# Autodesk Inventor assembly: Krasser Roboter
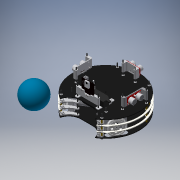
[picture p0: Inventor's stored thumbnail of the model, 180x180]
Saved by Autodesk Inventor 2018 (Build 220112000, 112)
## iProperties
Created: 2019-03-04
Part Number: Krasser Roboter
Material: Generisch
Document SubType Name: Assembly
Designer: RedBots
Mass: 1130.14 g
Surface Area: 3109.1 cm^2
Volume: 625.212 cm^3
Density: 1.80761 g/cm^3
Author: RedBots
## Documents named in this file (30)
- C:\Users\RedBots\Desktop\FinalRobot\Krasser Roboter.iam
- C:\Users\RedBots\Desktop\FinalRobot\Bodenplatine.ipt
- C:\Users\RedBots\Desktop\FinalRobot\motorhalterung 3.0.ipt
- C:\Users\RedBots\Desktop\FinalRobot\Gewindestange M3x100mm.ipt
- C:\Users\RedBots\Desktop\FinalRobot\Gewindestange M3x70mm.ipt
- C:\Users\RedBots\Desktop\FinalRobot\alu_ring_pesus.ipt
- C:\Users\RedBots\Desktop\FinalRobot\Fake Rad.ipt
- C:\Users\RedBots\Desktop\FinalRobot\Hauptplatine.ipt
- C:\Users\RedBots\Desktop\FinalRobot\Akku.ipt
- C:\Users\RedBots\Desktop\FinalRobot\Akkuhalterung.ipt
- C:\Users\RedBots\Desktop\FinalRobot\Schraube M3x8 SK.ipt
- C:\Users\RedBots\Desktop\FinalRobot\Motor\Motormaxon_PN_B7453F27107C.iam
- C:\Users\RedBots\Desktop\FinalRobot\Abstandshalter 15mm.ipt
- C:\Users\RedBots\Desktop\FinalRobot\LED 3mm.ipt
- C:\Users\RedBots\Desktop\FinalRobot\Halterung Lichtschranke rechts.ipt
- C:\Users\RedBots\Desktop\FinalRobot\Ball.ipt
- C:\Users\RedBots\Desktop\FinalRobot\Halterung Lichtschranke links.ipt
- C:\Users\RedBots\Desktop\FinalRobot\Abstandshalter 12mm.ipt
- C:\Users\RedBots\Desktop\FinalRobot\SRF08.ipt
- C:\Users\RedBots\Desktop\FinalRobot\US Halterung hinten.ipt
- C:\Users\RedBots\Desktop\FinalRobot\Pinhead 5.ipt
- C:\Users\RedBots\Desktop\FinalRobot\Schraube M3x8 LK.ipt
- C:\Users\RedBots\Desktop\FinalRobot\US Halterung rechts.ipt
- C:\Users\RedBots\Desktop\FinalRobot\US Halterung links.ipt
- C:\Users\RedBots\Desktop\FinalRobot\Pixy 2.iam
- C:\Users\RedBots\Desktop\FinalRobot\Pixy 2 Halterung.ipt
- C:\Users\RedBots\Desktop\FinalRobot\Abstandshalter US Sensor.ipt
- C:\Users\RedBots\Desktop\FinalRobot\Schraube M3x10 LK.ipt
- C:\Users\RedBots\Desktop\FinalRobot\Scheibe M3 Polyamid.ipt
- C:\Users\RedBots\Desktop\FinalRobot\Sicherungsmutter M3.ipt
## Components (131 placed, 30 different names)
1. Ball:1 — Passend:142, Passend:143
2. Abstandshalter US Sensor:1 — Passend:222, Passend:224, Passend:226
3. Abstandshalter US Sensor:2 — Passend:223, Passend:225
4. Bodenplatine:1 — Passend:16, Passend:17, Fluchtend:1, Fluchtend:2, Passend:18, Passend:19, Passend:20, Fluchtend:3, Fluchtend:4, Passend:21, Passend:22, Passend:23, Fluchtend:5, Fluchtend:6, Passend:24, Passend:25, Passend:26, Passend:27, Passend:28, Passend:29, Passend:30, Passend:31, Passend:32, Fluchtend:7, Fluchtend:8, Fluchtend:9, Fluchtend:10, Fluchtend:11, Fluchtend:12, Fluchtend:13, Fluchtend:14, Passend:100, Passend:102, Passend:105, Passend:106, Passend:143, Passend:157, Passend:158, Passend:262, Passend:263, Passend:264, Passend:265, Passend:266, Passend:267, Passend:268, Passend:269, Passend:270, Passend:271, Passend:272, Passend:273, Passend:274, Passend:275
5. Hauptplatine:1 — Passend:48, Passend:49, Passend:50, Passend:53, Passend:54, Passend:61, Passend:63, Passend:168, Passend:181, Passend:202, Passend:210, Passend:238, Passend:239, Passend:240, Passend:241, Passend:242, Passend:243, Passend:244, Passend:245, Passend:246, Passend:247, Passend:304
6. Gewindestange M3x100mm:1 — Passend:15, Passend:22, Fluchtend:6, Passend:169, Passend:233, Passend:255, Passend:284
7. Gewindestange M3x100mm:2 — Passend:14, Passend:23, Fluchtend:5, Passend:167, Passend:232, Passend:254, Passend:281
8. Gewindestange M3x100mm:8 — Passend:28, Fluchtend:8, Passend:62, Passend:128, Passend:137, Passend:140, Passend:209, Passend:250, Passend:293
9. Gewindestange M3x100mm:11 — Passend:26, Fluchtend:9, Passend:60, Passend:130, Passend:134, Passend:138, Passend:208, Passend:261, Passend:276
10. Gewindestange M3x100mm:12 — Passend:13, Passend:17, Fluchtend:2, Passend:179, Passend:235, Passend:258, Passend:292
11. Gewindestange M3x70mm:2 — Passend:12, Passend:16, Fluchtend:1, Passend:259, Passend:299
12. Gewindestange M3x100mm:14 — Passend:11, Passend:20, Fluchtend:3, Passend:203, Passend:229, Passend:251, Passend:278
13. Gewindestange M3x70mm:9 — Passend:10, Passend:19, Fluchtend:4, Passend:228, Passend:249, Passend:296
14. Gewindestange M3x70mm:1 — Passend:25, Fluchtend:10, Passend:33, Passend:36, Passend:49, Passend:86, Passend:87, Passend:112, Passend:131, Passend:135, Passend:139, Passend:234, Passend:260, Passend:298
15. Gewindestange M3x70mm:10 — Passend:29, Fluchtend:7, Passend:34, Passend:37, Passend:50, Passend:92, Passend:93, Passend:113, Passend:129, Passend:136, Passend:141, Passend:227, Passend:248, Passend:300
16. Gewindestange M3x100mm:15 — Passend:30, Fluchtend:14, Passend:94, Passend:95, Passend:114, Passend:204, Passend:230, Passend:252, Passend:280
17. Gewindestange M3x70mm:5 — Passend:32, Fluchtend:12, Passend:90, Passend:91, Passend:116, Passend:237, Passend:256, Passend:288
18. Gewindestange M3x70mm:6 — Passend:31, Fluchtend:13, Passend:96, Passend:97, Passend:117, Passend:231, Passend:253, Passend:285
19. Gewindestange M3x100mm:13 — Passend:27, Fluchtend:11, Passend:88, Passend:89, Passend:115, Passend:180, Passend:236, Passend:257, Passend:289
20. Ring unten — Passend:33, Passend:34, Passend:101, Passend:103, Passend:104, Passend:107, Passend:110, Passend:156, Passend:159
21. Ring oben — Passend:36, Passend:37, Passend:111, Passend:118, Passend:119, Passend:120, Passend:121, Passend:132, Passend:133
22. Fake Rad:1 — Tangential:2, Passend:75, Fluchtend:23
23. Fake Rad:2 — Tangential:1, Passend:70, Fluchtend:22
24. Fake Rad:3 — Passend:76, Fluchtend:24
25. Akku:1 — Passend:59, Passend:64, Fluchtend:18
26. Akkuhalterung:1 — Passend:54, Passend:62, Passend:63
27. Akkuhalterung:2 — Passend:53, Passend:59, Passend:60, Passend:61, Passend:64, Fluchtend:18
28. Motormaxon_PN_B7453F27107C:3 [sub-assembly] — Passend:68, Passend:69, Passend:70, Fluchtend:22, Passend:85
29. Motormaxon_PN_B7453F27107C:1 [sub-assembly] — Passend:71, Passend:72, Passend:75, Fluchtend:23, Passend:84
30. Motormaxon_PN_B7453F27107C:2 [sub-assembly] — Passend:73, Passend:74, Passend:76, Fluchtend:24, Passend:80, Passend:81, Passend:82, Passend:83
31. Abstandshalter 12mm:3 — Passend:86, Passend:98
32. Abstandshalter 12mm:2 — Passend:87, Passend:99
33. Abstandshalter 12mm:5 — Passend:93, Passend:109
34. Abstandshalter 12mm:6 — Passend:92, Passend:108, Passend:110
35. Abstandshalter 12mm:1 — Passend:112, Passend:122
36. Abstandshalter 12mm:4 — Passend:113, Passend:123
37. Abstandshalter 15mm:3 — Passend:97, Passend:104
38. Abstandshalter 15mm:4 — Passend:95, Passend:107, Passend:111
39. Abstandshalter 15mm:5 — Passend:96, Passend:105
40. Abstandshalter 15mm:6 — Passend:94, Passend:106
41. Abstandshalter 15mm:7 — Passend:88, Passend:101
42. Abstandshalter 15mm:8 — Passend:89, Passend:100
43. Abstandshalter 15mm:9 — Passend:90, Passend:102
44. Abstandshalter 15mm:10 — Passend:91, Passend:103
45. Abstandshalter 15mm:14 — Passend:115, Passend:121
46. Abstandshalter 15mm:16 — Passend:114, Passend:119
47. Abstandshalter 15mm:17 — Passend:116, Passend:120
48. Abstandshalter 15mm:18 — Passend:117, Passend:118
49. Halterung Lichtschranke links:1 — Passend:130, Passend:131, Passend:132, Passend:144, Passend:145, Passend:122
50. Halterung Lichtschranke links:2 — Passend:134, Passend:135, Passend:146, Passend:154, Passend:156, Passend:99
51. Halterung Lichtschranke rechts:2 — Passend:136, Passend:137, Passend:149, Passend:152, Passend:159, Passend:109
52. Halterung Lichtschranke links:3 — Passend:138, Passend:139, Passend:147, Passend:155, Passend:157, Passend:98
53. Halterung Lichtschranke rechts:3 — Passend:140, Passend:141, Passend:150, Passend:153, Passend:158, Passend:108
54. Halterung Lichtschranke rechts:1 — Passend:128, Passend:129, Passend:133, Passend:148, Passend:151, Passend:123
55. LED 3mm:1 — Passend:144, Passend:145
56. LED 3mm:2 — Passend:150, Passend:153
57. LED 3mm:3 — Passend:149, Passend:152
58. LED 3mm:4 — Passend:147, Passend:155
59. LED 3mm:5 — Passend:146, Passend:154
60. LED 3mm:6 — Passend:148, Passend:151
61. Schraube M3x10 LK:3
62. Schraube M3x10 LK:2
63. Schraube M3x10 LK:1
64. Pixy 2 Halterung:1 — Passend:208, Passend:209, Passend:210, Passend:212, Passend:213, Passend:214, Passend:215
65. Pixy 2:2 [sub-assembly] — Passend:212, Passend:213, Passend:214, Passend:215
66. Scheibe M3 Polyamid:1 — Passend:236, Passend:240
67. Scheibe M3 Polyamid:2 — Passend:235, Passend:239
68. Scheibe M3 Polyamid:3 — Passend:227, Passend:243
69. Scheibe M3 Polyamid:4 — Passend:234, Passend:238
70. Scheibe M3 Polyamid:6 — Passend:237, Passend:304
71. Scheibe M3 Polyamid:7 — Passend:233, Passend:247
72. Scheibe M3 Polyamid:8 — Passend:232, Passend:245
73. Scheibe M3 Polyamid:9 — Passend:231, Passend:246
74. Scheibe M3 Polyamid:10 — Passend:228, Passend:241
75. Scheibe M3 Polyamid:11 — Passend:229, Passend:242
76. Scheibe M3 Polyamid:12 — Passend:230, Passend:244
77. Scheibe M3 Polyamid:13 — Passend:251, Passend:265, Passend:279
78. Scheibe M3 Polyamid:14 — Passend:256, Passend:270, Passend:291
79. Scheibe M3 Polyamid:15 — Passend:248, Passend:262, Passend:303
80. Scheibe M3 Polyamid:16 — Passend:249, Passend:263, Passend:297
81. Scheibe M3 Polyamid:17 — Passend:260, Passend:275, Passend:301
82. Scheibe M3 Polyamid:18 — Passend:261, Passend:273, Passend:277
83. Scheibe M3 Polyamid:19 — Passend:258, Passend:272, Passend:295
84. Scheibe M3 Polyamid:20 — Passend:254, Passend:268, Passend:283
85. Scheibe M3 Polyamid:21 — Passend:255, Passend:269, Passend:286
86. Scheibe M3 Polyamid:22 — Passend:253, Passend:267, Passend:287
87. Scheibe M3 Polyamid:23 — Passend:259, Passend:274, Passend:302
88. Scheibe M3 Polyamid:24 — Passend:257, Passend:271, Passend:290
89. Scheibe M3 Polyamid:25 — Passend:252, Passend:266, Passend:282
90. Scheibe M3 Polyamid:26 — Passend:250, Passend:264, Passend:294
91. Sicherungsmutter M3:1 — Passend:288, Passend:291
92. Sicherungsmutter M3:2 — Passend:289, Passend:290
93. Sicherungsmutter M3:3 — Passend:278, Passend:279
94. Sicherungsmutter M3:4 — Passend:285, Passend:287
95. Sicherungsmutter M3:5 — Passend:284, Passend:286
96. Sicherungsmutter M3:6 — Passend:276, Passend:277
97. Sicherungsmutter M3:7 — Passend:280, Passend:282
98. Sicherungsmutter M3:8 — Passend:281, Passend:283
99. Sicherungsmutter M3:9 — Passend:296, Passend:297
100. Sicherungsmutter M3:10 — Passend:293, Passend:294
101. Sicherungsmutter M3:11 — Passend:292, Passend:295
102. Sicherungsmutter M3:12 — Passend:298, Passend:301
103. Sicherungsmutter M3:13 — Passend:299, Passend:302
104. Sicherungsmutter M3:14 — Passend:300, Passend:303
105. Schraube M3x8 SK:1 — Fluchtend:19, Passend:67
106. Schraube M3x8 SK:2 — Fluchtend:20, Passend:66
107. Schraube M3x8 SK:3 — Fluchtend:21, Passend:65
108. motorhalterung 3.0:1 — Passend:12, Passend:13, Passend:18, Fluchtend:19, Fluchtend:20, Fluchtend:21, Passend:65, Passend:66, Passend:67, Passend:71, Passend:72, Passend:84
109. motorhalterung 3.0:2 — Passend:14, Passend:15, Passend:24, Passend:68, Passend:69, Passend:77, Passend:78, Passend:79, Fluchtend:25, Fluchtend:26, Fluchtend:27, Passend:85
110. Schraube M3x8 SK:4 — Passend:77, Fluchtend:26
111. Schraube M3x8 SK:5 — Passend:78, Fluchtend:27
112. Schraube M3x8 SK:6 — Passend:79, Fluchtend:25
113. motorhalterung 3.0:3 — Passend:10, Passend:11, Passend:21, Passend:48, Passend:73, Passend:74, Passend:83, Fluchtend:28, Fluchtend:29, Fluchtend:30
114. Schraube M3x8 SK:7 — Passend:81, Fluchtend:28
115. Schraube M3x8 SK:8 — Passend:82, Fluchtend:30
116. Schraube M3x8 SK:9 — Passend:80, Fluchtend:29
117. Pinhead 5:1 — Passend:164, Passend:165, Passend:166
118. SRF08:3 — Passend:164, Passend:165, Passend:166, Passend:170, Passend:171, Passend:172, Passend:173, Passend:174, Passend:175, Passend:224, Passend:225
119. US Halterung hinten:1 — Passend:167, Passend:168, Passend:169, Passend:170, Passend:171, Passend:226
120. Schraube M3x8 LK:1 — Passend:173, Passend:174, Passend:223
121. Schraube M3x8 LK:2 — Passend:172, Passend:175, Passend:222
122. SRF08:2 — Passend:182, Passend:183, Passend:184, Passend:185, Passend:186, Passend:187, Passend:188, Passend:189
123. US Halterung rechts:1 — Passend:179, Passend:180, Passend:181, Passend:182, Passend:190, Passend:191
124. Pinhead 5:2 — Passend:183, Passend:184, Passend:185
125. Schraube M3x8 LK:3 — Passend:186, Passend:188, Passend:191
126. Schraube M3x8 LK:4 — Passend:187, Passend:189, Passend:190
127. SRF08:1 — Passend:195, Passend:196, Passend:197, Passend:198, Passend:199, Passend:200, Passend:201, Passend:205
128. Pinhead 5:3 — Passend:195, Passend:196, Passend:197
129. Schraube M3x8 LK:5 — Passend:199, Passend:201, Passend:207
130. Schraube M3x8 LK:6 — Passend:198, Passend:200, Passend:206
131. US Halterung links:1 — Passend:202, Passend:203, Passend:204, Passend:205, Passend:206, Passend:207
## Relationships (292: Mate 263, Flush 27, Tangent 2)
- Passend:10 [Mate]: Gewindestange M3x70mm:9 ↔ motorhalterung 3.0:3
- Passend:11 [Mate]: Gewindestange M3x100mm:14 ↔ motorhalterung 3.0:3
- Passend:12 [Mate]: Gewindestange M3x70mm:2 ↔ motorhalterung 3.0:1
- Passend:13 [Mate]: Gewindestange M3x100mm:12 ↔ motorhalterung 3.0:1
- Passend:14 [Mate]: Gewindestange M3x100mm:2 ↔ motorhalterung 3.0:2
- Passend:15 [Mate]: Gewindestange M3x100mm:1 ↔ motorhalterung 3.0:2
- Passend:16 [Mate]: Bodenplatine:1 ↔ Gewindestange M3x70mm:2
- Passend:17 [Mate]: Bodenplatine:1 ↔ Gewindestange M3x100mm:12
- Fluchtend:1 [Flush] (-5 mm): Bodenplatine:1 ↔ Gewindestange M3x70mm:2
- Fluchtend:2 [Flush] (-5 mm): Bodenplatine:1 ↔ Gewindestange M3x100mm:12
- Passend:18 [Mate]: Bodenplatine:1 ↔ motorhalterung 3.0:1
- Passend:19 [Mate]: Bodenplatine:1 ↔ Gewindestange M3x70mm:9
- Passend:20 [Mate]: Bodenplatine:1 ↔ Gewindestange M3x100mm:14
- Fluchtend:3 [Flush] (-5 mm): Bodenplatine:1 ↔ Gewindestange M3x100mm:14
- Fluchtend:4 [Flush] (5 mm): Bodenplatine:1 ↔ Gewindestange M3x70mm:9
- Passend:21 [Mate]: Bodenplatine:1 ↔ motorhalterung 3.0:3
- Passend:22 [Mate]: Bodenplatine:1 ↔ Gewindestange M3x100mm:1
- Passend:23 [Mate]: Bodenplatine:1 ↔ Gewindestange M3x100mm:2
- Fluchtend:5 [Flush] (-5 mm): Bodenplatine:1 ↔ Gewindestange M3x100mm:2
- Fluchtend:6 [Flush] (5 mm): Bodenplatine:1 ↔ Gewindestange M3x100mm:1
- Passend:24 [Mate]: Bodenplatine:1 ↔ motorhalterung 3.0:2
- Passend:25 [Mate]: Bodenplatine:1 ↔ Gewindestange M3x70mm:1
- Passend:26 [Mate]: Bodenplatine:1 ↔ Gewindestange M3x100mm:11
- Passend:27 [Mate]: Bodenplatine:1 ↔ Gewindestange M3x100mm:13
- Passend:28 [Mate]: Bodenplatine:1 ↔ Gewindestange M3x100mm:8
- Passend:29 [Mate]: Bodenplatine:1 ↔ Gewindestange M3x70mm:10
- Passend:30 [Mate]: Bodenplatine:1 ↔ Gewindestange M3x100mm:15
- Passend:31 [Mate]: Bodenplatine:1 ↔ Gewindestange M3x70mm:6
- Passend:32 [Mate]: Bodenplatine:1 ↔ Gewindestange M3x70mm:5
- Fluchtend:7 [Flush] (-5 mm): Bodenplatine:1 ↔ Gewindestange M3x70mm:10
- Fluchtend:8 [Flush] (5 mm): Bodenplatine:1 ↔ Gewindestange M3x100mm:8
- Fluchtend:9 [Flush] (5 mm): Bodenplatine:1 ↔ Gewindestange M3x100mm:11
- Fluchtend:10 [Flush] (5 mm): Bodenplatine:1 ↔ Gewindestange M3x70mm:1
- Fluchtend:11 [Flush] (-5 mm): Bodenplatine:1 ↔ Gewindestange M3x100mm:13
- Fluchtend:12 [Flush] (-5 mm): Bodenplatine:1 ↔ Gewindestange M3x70mm:5
- Fluchtend:13 [Flush] (-5 mm): Bodenplatine:1 ↔ Gewindestange M3x70mm:6
- Fluchtend:14 [Flush] (-5 mm): Bodenplatine:1 ↔ Gewindestange M3x100mm:15
- Passend:33 [Mate]: Gewindestange M3x70mm:1 ↔ Ring unten
- Passend:34 [Mate]: Gewindestange M3x70mm:10 ↔ Ring unten
- Passend:36 [Mate]: Gewindestange M3x70mm:1 ↔ Ring oben
- Passend:37 [Mate]: Gewindestange M3x70mm:10 ↔ Ring oben
- Passend:48 [Mate]: Hauptplatine:1 ↔ motorhalterung 3.0:3
- Passend:49 [Mate]: Hauptplatine:1 ↔ Gewindestange M3x70mm:1
- Passend:50 [Mate]: Hauptplatine:1 ↔ Gewindestange M3x70mm:10
- Passend:53 [Mate]: Hauptplatine:1 ↔ Akkuhalterung:2
- Passend:54 [Mate]: Hauptplatine:1 ↔ Akkuhalterung:1
- Passend:59 [Mate]: Akku:1 ↔ Akkuhalterung:2
- Passend:60 [Mate]: Gewindestange M3x100mm:11 ↔ Akkuhalterung:2
- Passend:61 [Mate]: Hauptplatine:1 ↔ Akkuhalterung:2
- Passend:62 [Mate]: Gewindestange M3x100mm:8 ↔ Akkuhalterung:1
- Passend:63 [Mate]: Hauptplatine:1 ↔ Akkuhalterung:1
- Tangential:1: Fake Rad:2
- Tangential:2: Fake Rad:1
- Passend:64 [Mate] (1.5 mm): Akku:1 ↔ Akkuhalterung:2
- Fluchtend:18 [Flush]: Akku:1 ↔ Akkuhalterung:2
- Fluchtend:19 [Flush]: Schraube M3x8 SK:1 ↔ motorhalterung 3.0:1
- Fluchtend:20 [Flush]: Schraube M3x8 SK:2 ↔ motorhalterung 3.0:1
- Fluchtend:21 [Flush]: Schraube M3x8 SK:3 ↔ motorhalterung 3.0:1
- Passend:65 [Mate]: Schraube M3x8 SK:3 ↔ motorhalterung 3.0:1
- Passend:66 [Mate]: Schraube M3x8 SK:2 ↔ motorhalterung 3.0:1
- Passend:67 [Mate]: Schraube M3x8 SK:1 ↔ motorhalterung 3.0:1
- Passend:68 [Mate]: Motormaxon_PN_B7453F27107C:3 ↔ motorhalterung 3.0:2
- Passend:69 [Mate]: Motormaxon_PN_B7453F27107C:3 ↔ motorhalterung 3.0:2
- Passend:70 [Mate]: Fake Rad:2 ↔ Motormaxon_PN_B7453F27107C:3
- Fluchtend:22 [Flush] (-0.5 mm): Fake Rad:2 ↔ Motormaxon_PN_B7453F27107C:3
- Passend:71 [Mate]: Motormaxon_PN_B7453F27107C:1 ↔ motorhalterung 3.0:1
- Passend:72 [Mate]: Motormaxon_PN_B7453F27107C:1 ↔ motorhalterung 3.0:1
- Passend:73 [Mate]: Motormaxon_PN_B7453F27107C:2 ↔ motorhalterung 3.0:3
- Passend:74 [Mate]: Motormaxon_PN_B7453F27107C:2 ↔ motorhalterung 3.0:3
- Passend:75 [Mate]: Fake Rad:1 ↔ Motormaxon_PN_B7453F27107C:1
- Fluchtend:23 [Flush] (0.5 mm): Fake Rad:1 ↔ Motormaxon_PN_B7453F27107C:1
- Passend:76 [Mate]: Fake Rad:3 ↔ Motormaxon_PN_B7453F27107C:2
- Fluchtend:24 [Flush] (-0.5 mm): Fake Rad:3 ↔ Motormaxon_PN_B7453F27107C:2
- Passend:77 [Mate]: motorhalterung 3.0:2 ↔ Schraube M3x8 SK:4
- Passend:78 [Mate]: motorhalterung 3.0:2 ↔ Schraube M3x8 SK:5
- Passend:79 [Mate]: motorhalterung 3.0:2 ↔ Schraube M3x8 SK:6
- Fluchtend:25 [Flush]: motorhalterung 3.0:2 ↔ Schraube M3x8 SK:6
- Fluchtend:26 [Flush]: motorhalterung 3.0:2 ↔ Schraube M3x8 SK:4
- Fluchtend:27 [Flush]: motorhalterung 3.0:2 ↔ Schraube M3x8 SK:5
- Passend:80 [Mate]: Motormaxon_PN_B7453F27107C:2 ↔ Schraube M3x8 SK:9
- Passend:81 [Mate]: Motormaxon_PN_B7453F27107C:2 ↔ Schraube M3x8 SK:7
- Passend:82 [Mate]: Motormaxon_PN_B7453F27107C:2 ↔ Schraube M3x8 SK:8
- Passend:83 [Mate]: Motormaxon_PN_B7453F27107C:2 ↔ motorhalterung 3.0:3
- Fluchtend:28 [Flush]: motorhalterung 3.0:3 ↔ Schraube M3x8 SK:7
- Fluchtend:29 [Flush]: motorhalterung 3.0:3 ↔ Schraube M3x8 SK:9
- Fluchtend:30 [Flush]: motorhalterung 3.0:3 ↔ Schraube M3x8 SK:8
- Passend:84 [Mate]: Motormaxon_PN_B7453F27107C:1 ↔ motorhalterung 3.0:1
- Passend:85 [Mate]: Motormaxon_PN_B7453F27107C:3 ↔ motorhalterung 3.0:2
- Passend:86 [Mate]: Gewindestange M3x70mm:1 ↔ Abstandshalter 12mm:3
- Passend:87 [Mate]: Gewindestange M3x70mm:1 ↔ Abstandshalter 12mm:2
- Passend:88 [Mate]: Gewindestange M3x100mm:13 ↔ Abstandshalter 15mm:7
- Passend:89 [Mate]: Gewindestange M3x100mm:13 ↔ Abstandshalter 15mm:8
- Passend:90 [Mate]: Gewindestange M3x70mm:5 ↔ Abstandshalter 15mm:9
- Passend:91 [Mate]: Gewindestange M3x70mm:5 ↔ Abstandshalter 15mm:10
- Passend:92 [Mate]: Gewindestange M3x70mm:10 ↔ Abstandshalter 12mm:6
- Passend:93 [Mate]: Gewindestange M3x70mm:10 ↔ Abstandshalter 12mm:5
- Passend:94 [Mate]: Gewindestange M3x100mm:15 ↔ Abstandshalter 15mm:6
- Passend:95 [Mate]: Gewindestange M3x100mm:15 ↔ Abstandshalter 15mm:4
- Passend:96 [Mate]: Gewindestange M3x70mm:6 ↔ Abstandshalter 15mm:5
- Passend:97 [Mate]: Gewindestange M3x70mm:6 ↔ Abstandshalter 15mm:3
- Passend:98 [Mate]: Abstandshalter 12mm:3 ↔ Halterung Lichtschranke links:3
- Passend:99 [Mate]: Abstandshalter 12mm:2 ↔ Halterung Lichtschranke links:2
- Passend:100 [Mate]: Bodenplatine:1 ↔ Abstandshalter 15mm:8
- Passend:101 [Mate]: Ring unten ↔ Abstandshalter 15mm:7
- Passend:102 [Mate]: Bodenplatine:1 ↔ Abstandshalter 15mm:9
- Passend:103 [Mate]: Ring unten ↔ Abstandshalter 15mm:10
- Passend:104 [Mate]: Ring unten ↔ Abstandshalter 15mm:3
- Passend:105 [Mate]: Bodenplatine:1 ↔ Abstandshalter 15mm:5
- Passend:106 [Mate]: Bodenplatine:1 ↔ Abstandshalter 15mm:6
- Passend:107 [Mate]: Ring unten ↔ Abstandshalter 15mm:4
- Passend:108 [Mate]: Abstandshalter 12mm:6 ↔ Halterung Lichtschranke rechts:3
- Passend:109 [Mate]: Abstandshalter 12mm:5 ↔ Halterung Lichtschranke rechts:2
- Passend:110 [Mate]: Ring unten ↔ Abstandshalter 12mm:6
- Passend:111 [Mate]: Ring oben ↔ Abstandshalter 15mm:4
- Passend:112 [Mate]: Gewindestange M3x70mm:1 ↔ Abstandshalter 12mm:1
- Passend:113 [Mate]: Gewindestange M3x70mm:10 ↔ Abstandshalter 12mm:4
- Passend:114 [Mate]: Gewindestange M3x100mm:15 ↔ Abstandshalter 15mm:16
- Passend:115 [Mate]: Gewindestange M3x100mm:13 ↔ Abstandshalter 15mm:14
- Passend:116 [Mate]: Gewindestange M3x70mm:5 ↔ Abstandshalter 15mm:17
- Passend:117 [Mate]: Gewindestange M3x70mm:6 ↔ Abstandshalter 15mm:18
- Passend:118 [Mate]: Ring oben ↔ Abstandshalter 15mm:18
- Passend:119 [Mate]: Ring oben ↔ Abstandshalter 15mm:16
- Passend:120 [Mate]: Ring oben ↔ Abstandshalter 15mm:17
- Passend:121 [Mate]: Ring oben ↔ Abstandshalter 15mm:14
- Passend:122 [Mate]: Abstandshalter 12mm:1 ↔ Halterung Lichtschranke links:1
- Passend:123 [Mate]: Abstandshalter 12mm:4 ↔ Halterung Lichtschranke rechts:1
- Passend:128 [Mate]: Gewindestange M3x100mm:8 ↔ Halterung Lichtschranke rechts:1
- Passend:129 [Mate]: Gewindestange M3x70mm:10 ↔ Halterung Lichtschranke rechts:1
- Passend:130 [Mate]: Gewindestange M3x100mm:11 ↔ Halterung Lichtschranke links:1
- Passend:131 [Mate]: Gewindestange M3x70mm:1 ↔ Halterung Lichtschranke links:1
- Passend:132 [Mate]: Ring oben ↔ Halterung Lichtschranke links:1
- Passend:133 [Mate]: Ring oben ↔ Halterung Lichtschranke rechts:1
- Passend:134 [Mate]: Gewindestange M3x100mm:11 ↔ Halterung Lichtschranke links:2
- Passend:135 [Mate]: Gewindestange M3x70mm:1 ↔ Halterung Lichtschranke links:2
- Passend:136 [Mate]: Gewindestange M3x70mm:10 ↔ Halterung Lichtschranke rechts:2
- Passend:137 [Mate]: Gewindestange M3x100mm:8 ↔ Halterung Lichtschranke rechts:2
- Passend:138 [Mate]: Gewindestange M3x100mm:11 ↔ Halterung Lichtschranke links:3
- Passend:139 [Mate]: Gewindestange M3x70mm:1 ↔ Halterung Lichtschranke links:3
- Passend:140 [Mate]: Gewindestange M3x100mm:8 ↔ Halterung Lichtschranke rechts:3
- Passend:141 [Mate]: Gewindestange M3x70mm:10 ↔ Halterung Lichtschranke rechts:3
- Passend:142 [Mate] (37 mm): Ball:1
- Passend:143 [Mate] (37 mm): Ball:1 ↔ Bodenplatine:1
- Passend:144 [Mate]: Halterung Lichtschranke links:1 ↔ LED 3mm:1
- Passend:145 [Mate]: Halterung Lichtschranke links:1 ↔ LED 3mm:1
- Passend:146 [Mate]: Halterung Lichtschranke links:2 ↔ LED 3mm:5
- Passend:147 [Mate]: Halterung Lichtschranke links:3 ↔ LED 3mm:4
- Passend:148 [Mate]: Halterung Lichtschranke rechts:1 ↔ LED 3mm:6
- Passend:149 [Mate]: Halterung Lichtschranke rechts:2 ↔ LED 3mm:3
- Passend:150 [Mate]: Halterung Lichtschranke rechts:3 ↔ LED 3mm:2
- Passend:151 [Mate]: Halterung Lichtschranke rechts:1 ↔ LED 3mm:6
- Passend:152 [Mate]: Halterung Lichtschranke rechts:2 ↔ LED 3mm:3
- Passend:153 [Mate]: Halterung Lichtschranke rechts:3 ↔ LED 3mm:2
- Passend:154 [Mate]: Halterung Lichtschranke links:2 ↔ LED 3mm:5
- Passend:155 [Mate]: Halterung Lichtschranke links:3 ↔ LED 3mm:4
- Passend:156 [Mate]: Ring unten ↔ Halterung Lichtschranke links:2
- Passend:157 [Mate]: Bodenplatine:1 ↔ Halterung Lichtschranke links:3
- Passend:158 [Mate]: Bodenplatine:1 ↔ Halterung Lichtschranke rechts:3
- Passend:159 [Mate]: Ring unten ↔ Halterung Lichtschranke rechts:2
- Passend:164 [Mate]: Pinhead 5:1 ↔ SRF08:3
- Passend:165 [Mate]: Pinhead 5:1 ↔ SRF08:3
- Passend:166 [Mate]: Pinhead 5:1 ↔ SRF08:3
- Passend:167 [Mate]: Gewindestange M3x100mm:2 ↔ US Halterung hinten:1
- Passend:168 [Mate] (10 mm): Hauptplatine:1 ↔ US Halterung hinten:1
- Passend:169 [Mate]: Gewindestange M3x100mm:1 ↔ US Halterung hinten:1
- Passend:170 [Mate]: SRF08:3 ↔ US Halterung hinten:1
- Passend:171 [Mate]: SRF08:3 ↔ US Halterung hinten:1
- Passend:172 [Mate]: SRF08:3 ↔ Schraube M3x8 LK:2
- Passend:173 [Mate]: SRF08:3 ↔ Schraube M3x8 LK:1
- Passend:174 [Mate]: SRF08:3 ↔ Schraube M3x8 LK:1
- Passend:175 [Mate]: SRF08:3 ↔ Schraube M3x8 LK:2
- Passend:179 [Mate]: Gewindestange M3x100mm:12 ↔ US Halterung rechts:1
- Passend:180 [Mate]: Gewindestange M3x100mm:13 ↔ US Halterung rechts:1
- Passend:181 [Mate] (10 mm): Hauptplatine:1 ↔ US Halterung rechts:1
- Passend:182 [Mate]: SRF08:2 ↔ US Halterung rechts:1
- Passend:183 [Mate]: SRF08:2 ↔ Pinhead 5:2
- Passend:184 [Mate]: SRF08:2 ↔ Pinhead 5:2
- Passend:185 [Mate]: SRF08:2 ↔ Pinhead 5:2
- Passend:186 [Mate]: SRF08:2 ↔ Schraube M3x8 LK:3
- Passend:187 [Mate]: SRF08:2 ↔ Schraube M3x8 LK:4
- Passend:188 [Mate]: SRF08:2 ↔ Schraube M3x8 LK:3
- Passend:189 [Mate]: SRF08:2 ↔ Schraube M3x8 LK:4
- Passend:190 [Mate]: US Halterung rechts:1 ↔ Schraube M3x8 LK:4
- Passend:191 [Mate]: US Halterung rechts:1 ↔ Schraube M3x8 LK:3
- Passend:195 [Mate]: SRF08:1 ↔ Pinhead 5:3
- Passend:196 [Mate]: SRF08:1 ↔ Pinhead 5:3
- Passend:197 [Mate]: SRF08:1 ↔ Pinhead 5:3
- Passend:198 [Mate]: SRF08:1 ↔ Schraube M3x8 LK:6
- Passend:199 [Mate]: SRF08:1 ↔ Schraube M3x8 LK:5
- Passend:200 [Mate]: SRF08:1 ↔ Schraube M3x8 LK:6
- Passend:201 [Mate]: SRF08:1 ↔ Schraube M3x8 LK:5
- Passend:202 [Mate] (10 mm): Hauptplatine:1 ↔ US Halterung links:1
- Passend:203 [Mate]: Gewindestange M3x100mm:14 ↔ US Halterung links:1
- Passend:204 [Mate]: Gewindestange M3x100mm:15 ↔ US Halterung links:1
- Passend:205 [Mate]: SRF08:1 ↔ US Halterung links:1
- Passend:206 [Mate]: Schraube M3x8 LK:6 ↔ US Halterung links:1
- Passend:207 [Mate]: Schraube M3x8 LK:5 ↔ US Halterung links:1
- Passend:208 [Mate]: Gewindestange M3x100mm:11 ↔ Pixy 2 Halterung:1
- Passend:209 [Mate]: Gewindestange M3x100mm:8 ↔ Pixy 2 Halterung:1
- Passend:210 [Mate] (10 mm): Hauptplatine:1 ↔ Pixy 2 Halterung:1
- Passend:212 [Mate]: Pixy 2 Halterung:1 ↔ Pixy 2:2
- Passend:213 [Mate]: Pixy 2 Halterung:1 ↔ Pixy 2:2
- Passend:214 [Mate]: Pixy 2 Halterung:1 ↔ Pixy 2:2
- Passend:215 [Mate]: Pixy 2 Halterung:1 ↔ Pixy 2:2
- [Mate]: Schraube M3x10 LK:1 ↔ Pixy 2 Halterung:1
- [Mate]: Schraube M3x10 LK:2 ↔ Pixy 2 Halterung:1
- [Mate]: Schraube M3x10 LK:3 ↔ Pixy 2 Halterung:1
- [Mate]: Schraube M3x10 LK:3 ↔ Pixy 2 Halterung:1
- [Mate]: Schraube M3x10 LK:2 ↔ Pixy 2 Halterung:1
- [Mate]: Schraube M3x10 LK:1 ↔ Pixy 2 Halterung:1
- Passend:222 [Mate]: Abstandshalter US Sensor:1 ↔ Schraube M3x8 LK:2
- Passend:223 [Mate]: Abstandshalter US Sensor:2 ↔ Schraube M3x8 LK:1
- Passend:224 [Mate]: Abstandshalter US Sensor:1 ↔ SRF08:3
- Passend:225 [Mate]: Abstandshalter US Sensor:2 ↔ SRF08:3
- Passend:226 [Mate]: Abstandshalter US Sensor:1 ↔ US Halterung hinten:1
- Passend:227 [Mate]: Gewindestange M3x70mm:10 ↔ Scheibe M3 Polyamid:3
- Passend:228 [Mate]: Gewindestange M3x70mm:9 ↔ Scheibe M3 Polyamid:10
- Passend:229 [Mate]: Gewindestange M3x100mm:14 ↔ Scheibe M3 Polyamid:11
- Passend:230 [Mate]: Gewindestange M3x100mm:15 ↔ Scheibe M3 Polyamid:12
- Passend:231 [Mate]: Gewindestange M3x70mm:6 ↔ Scheibe M3 Polyamid:9
- Passend:232 [Mate]: Gewindestange M3x100mm:2 ↔ Scheibe M3 Polyamid:8
- Passend:233 [Mate]: Gewindestange M3x100mm:1 ↔ Scheibe M3 Polyamid:7
- Passend:234 [Mate]: Gewindestange M3x70mm:1 ↔ Scheibe M3 Polyamid:4
- Passend:235 [Mate]: Gewindestange M3x100mm:12 ↔ Scheibe M3 Polyamid:2
- Passend:236 [Mate]: Gewindestange M3x100mm:13 ↔ Scheibe M3 Polyamid:1
- Passend:237 [Mate]: Gewindestange M3x70mm:5 ↔ Scheibe M3 Polyamid:6
- Passend:238 [Mate]: Hauptplatine:1 ↔ Scheibe M3 Polyamid:4
- Passend:239 [Mate]: Hauptplatine:1 ↔ Scheibe M3 Polyamid:2
- Passend:240 [Mate]: Hauptplatine:1 ↔ Scheibe M3 Polyamid:1
- Passend:241 [Mate]: Hauptplatine:1 ↔ Scheibe M3 Polyamid:10
- Passend:242 [Mate]: Hauptplatine:1 ↔ Scheibe M3 Polyamid:11
- Passend:243 [Mate]: Hauptplatine:1 ↔ Scheibe M3 Polyamid:3
- Passend:244 [Mate]: Hauptplatine:1 ↔ Scheibe M3 Polyamid:12
- Passend:245 [Mate]: Hauptplatine:1 ↔ Scheibe M3 Polyamid:8
- Passend:246 [Mate]: Hauptplatine:1 ↔ Scheibe M3 Polyamid:9
- Passend:247 [Mate]: Hauptplatine:1 ↔ Scheibe M3 Polyamid:7
- Passend:248 [Mate]: Gewindestange M3x70mm:10 ↔ Scheibe M3 Polyamid:15
- Passend:249 [Mate]: Gewindestange M3x70mm:9 ↔ Scheibe M3 Polyamid:16
- Passend:250 [Mate]: Gewindestange M3x100mm:8 ↔ Scheibe M3 Polyamid:26
- Passend:251 [Mate]: Gewindestange M3x100mm:14 ↔ Scheibe M3 Polyamid:13
- Passend:252 [Mate]: Gewindestange M3x100mm:15 ↔ Scheibe M3 Polyamid:25
- Passend:253 [Mate]: Gewindestange M3x70mm:6 ↔ Scheibe M3 Polyamid:22
- Passend:254 [Mate]: Gewindestange M3x100mm:2 ↔ Scheibe M3 Polyamid:20
- Passend:255 [Mate]: Gewindestange M3x100mm:1 ↔ Scheibe M3 Polyamid:21
- Passend:256 [Mate]: Gewindestange M3x70mm:5 ↔ Scheibe M3 Polyamid:14
- Passend:257 [Mate]: Gewindestange M3x100mm:13 ↔ Scheibe M3 Polyamid:24
- Passend:258 [Mate]: Gewindestange M3x100mm:12 ↔ Scheibe M3 Polyamid:19
- Passend:259 [Mate]: Gewindestange M3x70mm:2 ↔ Scheibe M3 Polyamid:23
- Passend:260 [Mate]: Gewindestange M3x70mm:1 ↔ Scheibe M3 Polyamid:17
- Passend:261 [Mate]: Gewindestange M3x100mm:11 ↔ Scheibe M3 Polyamid:18
- Passend:262 [Mate]: Bodenplatine:1 ↔ Scheibe M3 Polyamid:15
- Passend:263 [Mate]: Bodenplatine:1 ↔ Scheibe M3 Polyamid:16
- Passend:264 [Mate]: Bodenplatine:1 ↔ Scheibe M3 Polyamid:26
- Passend:265 [Mate]: Bodenplatine:1 ↔ Scheibe M3 Polyamid:13
- Passend:266 [Mate]: Bodenplatine:1 ↔ Scheibe M3 Polyamid:25
- Passend:267 [Mate]: Bodenplatine:1 ↔ Scheibe M3 Polyamid:22
- Passend:268 [Mate]: Bodenplatine:1 ↔ Scheibe M3 Polyamid:20
- Passend:269 [Mate]: Bodenplatine:1 ↔ Scheibe M3 Polyamid:21
- Passend:270 [Mate]: Bodenplatine:1 ↔ Scheibe M3 Polyamid:14
- Passend:271 [Mate]: Bodenplatine:1 ↔ Scheibe M3 Polyamid:24
- Passend:272 [Mate]: Bodenplatine:1 ↔ Scheibe M3 Polyamid:19
- Passend:273 [Mate]: Bodenplatine:1 ↔ Scheibe M3 Polyamid:18
- Passend:274 [Mate]: Bodenplatine:1 ↔ Scheibe M3 Polyamid:23
- Passend:275 [Mate]: Bodenplatine:1 ↔ Scheibe M3 Polyamid:17
- Passend:276 [Mate]: Gewindestange M3x100mm:11 ↔ Sicherungsmutter M3:6
- Passend:277 [Mate]: Scheibe M3 Polyamid:18 ↔ Sicherungsmutter M3:6
- Passend:278 [Mate]: Gewindestange M3x100mm:14 ↔ Sicherungsmutter M3:3
- Passend:279 [Mate]: Scheibe M3 Polyamid:13 ↔ Sicherungsmutter M3:3
- Passend:280 [Mate]: Gewindestange M3x100mm:15 ↔ Sicherungsmutter M3:7
- Passend:281 [Mate]: Gewindestange M3x100mm:2 ↔ Sicherungsmutter M3:8
- Passend:282 [Mate]: Scheibe M3 Polyamid:25 ↔ Sicherungsmutter M3:7
- Passend:283 [Mate]: Scheibe M3 Polyamid:20 ↔ Sicherungsmutter M3:8
- Passend:284 [Mate]: Gewindestange M3x100mm:1 ↔ Sicherungsmutter M3:5
- Passend:285 [Mate]: Gewindestange M3x70mm:6 ↔ Sicherungsmutter M3:4
- Passend:286 [Mate]: Scheibe M3 Polyamid:21 ↔ Sicherungsmutter M3:5
- Passend:287 [Mate]: Scheibe M3 Polyamid:22 ↔ Sicherungsmutter M3:4
- Passend:288 [Mate]: Gewindestange M3x70mm:5 ↔ Sicherungsmutter M3:1
- Passend:289 [Mate]: Gewindestange M3x100mm:13 ↔ Sicherungsmutter M3:2
- Passend:290 [Mate]: Scheibe M3 Polyamid:24 ↔ Sicherungsmutter M3:2
- Passend:291 [Mate]: Scheibe M3 Polyamid:14 ↔ Sicherungsmutter M3:1
- Passend:292 [Mate]: Gewindestange M3x100mm:12 ↔ Sicherungsmutter M3:11
- Passend:293 [Mate]: Gewindestange M3x100mm:8 ↔ Sicherungsmutter M3:10
- Passend:294 [Mate]: Scheibe M3 Polyamid:26 ↔ Sicherungsmutter M3:10
- Passend:295 [Mate]: Scheibe M3 Polyamid:19 ↔ Sicherungsmutter M3:11
- Passend:296 [Mate]: Gewindestange M3x70mm:9 ↔ Sicherungsmutter M3:9
- Passend:297 [Mate]: Scheibe M3 Polyamid:16 ↔ Sicherungsmutter M3:9
- Passend:298 [Mate]: Gewindestange M3x70mm:1 ↔ Sicherungsmutter M3:12
- Passend:299 [Mate]: Gewindestange M3x70mm:2 ↔ Sicherungsmutter M3:13
- Passend:300 [Mate]: Gewindestange M3x70mm:10 ↔ Sicherungsmutter M3:14
- Passend:301 [Mate]: Scheibe M3 Polyamid:17 ↔ Sicherungsmutter M3:12
- Passend:302 [Mate]: Scheibe M3 Polyamid:23 ↔ Sicherungsmutter M3:13
- Passend:303 [Mate]: Scheibe M3 Polyamid:15 ↔ Sicherungsmutter M3:14
- Passend:304 [Mate]: Hauptplatine:1 ↔ Scheibe M3 Polyamid:6
